# Autodesk Inventor assembly: Idler Front Tensioner-Unit [A]
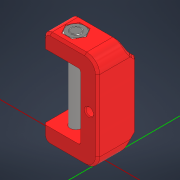
[picture p0: Inventor's stored thumbnail of the model, 180x180]
Saved by Autodesk Inventor 2022.2 (Build 262287010, 287A)
## iProperties
Created: 2022-03-14
Part Number: Idler Front Tensioner-Unit [A]
Document SubType Name: Assembly
Designer: sleib
Author: sleib
## Documents named in this file (5)
- C:\Users\sleib\Projekte\Voron-2\CAD\Inventor\Idler Front Tensioner-Unit [A].iam
- C:\Users\sleib\Projekte\Voron-2\CAD\Inventor\Idler Front Tensioner [A].ipt
- C:\Users\sleib\Projekte\Voron-2\CAD\Inventor\M3 Threaded Insert.ipt
- C:\Users\sleib\Projekte\Voron-2\CAD\Inventor\M5 Hexnut.ipt
- C:\Users\sleib\Projekte\Voron-2\CAD\Inventor\M5x40 SHCS.ipt
## Components (4 placed, 4 different names)
1. Idler Front Tensioner [A]:1 — Passend:1, Winkel:1, Passend:2, Passend:3, Passend:4, Fluchtend:1, Winkel:2, Passend:5, Passend:6, Passend:7, Passend:8
2. M3 Threaded Insert:1 — Passend:4, Fluchtend:1
3. M5 Hexnut:1 — Winkel:2, Passend:5, Passend:6
4. M5x40 SHCS:1 — Passend:7, Passend:8
## Relationships (11: Mate 8, Angle 2, Flush 1)
- Passend:1 [Mate]: Idler Front Tensioner [A]:1
- Winkel:1 [Angle] (-90 deg): Idler Front Tensioner [A]:1
- Passend:2 [Mate]: Idler Front Tensioner [A]:1
- Passend:3 [Mate]: Idler Front Tensioner [A]:1
- Passend:4 [Mate]: Idler Front Tensioner [A]:1 ↔ M3 Threaded Insert:1
- Fluchtend:1 [Flush]: Idler Front Tensioner [A]:1 ↔ M3 Threaded Insert:1
- Winkel:2 [Angle] (0 deg): Idler Front Tensioner [A]:1 ↔ M5 Hexnut:1
- Passend:5 [Mate]: Idler Front Tensioner [A]:1 ↔ M5 Hexnut:1
- Passend:6 [Mate]: Idler Front Tensioner [A]:1 ↔ M5 Hexnut:1
- Passend:7 [Mate]: Idler Front Tensioner [A]:1 ↔ M5x40 SHCS:1
- Passend:8 [Mate]: Idler Front Tensioner [A]:1 ↔ M5x40 SHCS:1
